# Autodesk Inventor assembly: PumpkinAssembly
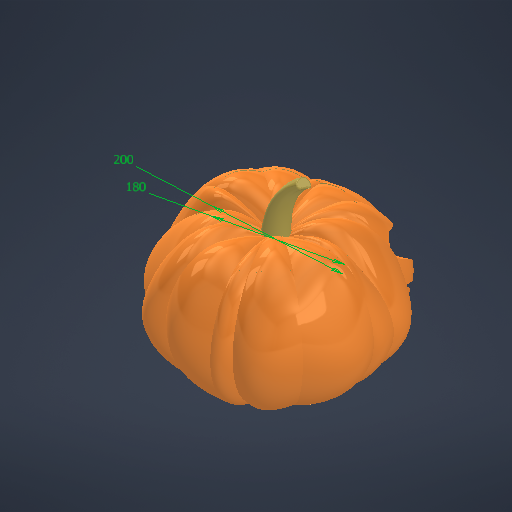
[picture p0: Inventor's stored thumbnail of the model, 512x512]
Saved by Autodesk Inventor 2025.1 (Build 291241020, 241B)
## iProperties
Created: 2024-09-28
Part Number: PumpkinAssembly
Document SubType Name: Assembly
Designer: brett
Author: brett
## Documents named in this file (3)
- C:\Users\brett\OneDrive\Desktop\Projects\Halloween Project\HalloweenProject\CAD Pumpkin\PumpkinAssembly.iam
- C:\Users\brett\OneDrive\Desktop\Projects\Halloween Project\HalloweenProject\CAD Pumpkin\Pumpkin.ipt
- C:\Users\brett\OneDrive\Desktop\Projects\Halloween Project\HalloweenProject\CAD Pumpkin\PumpkinTop.ipt
## Components (2 placed, 2 different names)
1. Pumpkin:1 — Rotational:1
2. PumpkinTop:1 — Rotational:1
## Relationships (1: RevoluteJoint 1)
- Rotational:1 [RevoluteJoint]: Pumpkin:1 ↔ PumpkinTop:1
